# Autodesk Inventor assembly: Spidey
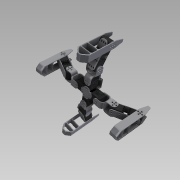
[picture p0: Inventor's stored thumbnail of the model, 180x180]
Saved by Autodesk Inventor 2014 (Build 180170000, 170)
## iProperties
Created: 2014-03-07
Part Number: Spidey
Document SubType Name: Assembly
Designer: Grégoire
Author: Grégoire
## Documents named in this file (10)
- C:\Users\Grégoire\Desktop\Spidey\3d\src\spidey.iam
- C:\Users\Grégoire\Desktop\Spidey\3d\src\models\motor.ipt
- C:\Users\Grégoire\Desktop\Spidey\3d\src\models\arm.ipt
- C:\Users\Grégoire\Desktop\Spidey\3d\src\models\counter_arm.ipt
- C:\Users\Grégoire\Desktop\Spidey\3d\src\parts\u.ipt
- C:\Users\Grégoire\Desktop\Spidey\3d\src\parts\side.ipt
- C:\Users\Grégoire\Desktop\Spidey\3d\src\parts\leg.ipt
- C:\Users\Grégoire\Desktop\Spidey\3d\src\parts\body.ipt
- C:\Users\Grégoire\Desktop\Spidey\3d\src\parts\body_with_fixations.ipt
- C:\Users\Grégoire\Desktop\Spidey\3d\src\parts\body_to_opencm.ipt
## Components (60 placed, 9 different names)
1. motor:4 — Placage:132, Placage:133, Placage:148, Placage:152
2. arm:4
3. counter_arm:4
4. u:3
5. u:4
6. motor:5
7. arm:5
8. counter_arm:5
9. side:3
10. side:4
11. motor:6
12. arm:6
13. counter_arm:6
14. leg:2
15. motor:7 — Placage:127, Placage:128, Placage:150, Placage:153, Placage:154
16. arm:7
17. counter_arm:7
18. u:5
19. u:6
20. motor:8
21. arm:8
22. counter_arm:8
23. side:5
24. side:6
25. motor:9
26. arm:9
27. counter_arm:9
28. leg:3
29. motor:10 — Placage:129, Placage:151, Placage:156, Placage:157
30. arm:10
31. counter_arm:10
32. u:7
33. u:8
34. motor:11
35. arm:11
36. counter_arm:11
37. side:7
38. side:8
39. motor:12
40. arm:12
41. counter_arm:12
42. leg:4
43. body:1 — Placage:127, Placage:128, Placage:129, Placage:130, Placage:131, Placage:132, Placage:133, Placage:148, Placage:165
44. body_with_fixations:1 — Placage:149, Placage:150, Placage:151, Placage:152, Placage:153, Placage:154, Placage:155, Placage:156, Placage:157, Placage:158, Placage:159, Placage:160, Placage:161, Placage:162, Placage:163
45. body_to_opencm:1 — Placage:158, Placage:162, Placage:163
46. body_to_opencm:2 — Placage:159, Placage:160, Placage:161
47. u:1 — Placage:7, Placage:8, Placage:9, Placage:14, Placage:15
48. u:2 — Placage:5, Placage:6, Placage:7, Placage:8, Placage:9, Placage:164
49. side:1 — Placage:19, Placage:20, Placage:21, Placage:26, Placage:27, Placage:28
50. side:2 — Placage:16, Placage:17, Placage:18
51. leg:1 — Placage:29, Placage:30
52. motor:1 — Placage:1, Placage:2, Placage:3, Placage:4, Placage:130, Placage:131, Placage:149, Placage:155
53. arm:1 — Placage:3, Placage:4, Placage:5, Placage:6
54. counter_arm:1 — Placage:1, Placage:2, Placage:164
55. motor:2 — Placage:16, Placage:17, Placage:18, Placage:19, Placage:20, Placage:21
56. arm:2 — Placage:15
57. counter_arm:2 — Placage:14
58. motor:3 — Placage:26, Placage:27, Placage:28
59. arm:3 — Placage:29, Placage:30
60. counter_arm:3
## Relationships (145: Mate 145)
- Placage:1 [Mate]: motor:1 ↔ counter_arm:1
- Placage:2 [Mate]: motor:1 ↔ counter_arm:1
- Placage:3 [Mate]: motor:1 ↔ arm:1
- Placage:4 [Mate]: motor:1 ↔ arm:1
- Placage:5 [Mate]: u:2 ↔ arm:1
- Placage:6 [Mate]: u:2 ↔ arm:1
- Placage:7 [Mate]: u:1 ↔ u:2
- Placage:8 [Mate]: u:1 ↔ u:2
- Placage:9 [Mate]: u:1 ↔ u:2
- [Mate]: motor:2 ↔ counter_arm:2
- [Mate]: motor:2 ↔ counter_arm:2
- [Mate]: motor:2 ↔ arm:2
- [Mate]: motor:2 ↔ arm:2
- Placage:14 [Mate]: u:1 ↔ counter_arm:2
- Placage:15 [Mate]: u:1 ↔ arm:2
- Placage:16 [Mate]: side:2 ↔ motor:2
- Placage:17 [Mate]: side:2 ↔ motor:2
- Placage:18 [Mate]: side:2 ↔ motor:2
- Placage:19 [Mate]: side:1 ↔ motor:2
- Placage:20 [Mate]: side:1 ↔ motor:2
- Placage:21 [Mate]: side:1 ↔ motor:2
- [Mate]: motor:3 ↔ counter_arm:3
- [Mate]: motor:3 ↔ counter_arm:3
- [Mate]: motor:3 ↔ arm:3
- [Mate]: motor:3 ↔ arm:3
- Placage:26 [Mate]: side:1 ↔ motor:3
- Placage:27 [Mate]: side:1 ↔ motor:3
- Placage:28 [Mate]: side:1 ↔ motor:3
- Placage:29 [Mate]: leg:1 ↔ arm:3
- Placage:30 [Mate]: leg:1 ↔ arm:3
- [Mate]: motor:4 ↔ counter_arm:4
- [Mate]: motor:4 ↔ counter_arm:4
- [Mate]: motor:4 ↔ arm:4
- [Mate]: motor:4 ↔ arm:4
- [Mate]: arm:4 ↔ u:4
- [Mate]: arm:4 ↔ u:4
- [Mate]: u:3 ↔ u:4
- [Mate]: u:3 ↔ u:4
- [Mate]: u:3 ↔ u:4
- [Mate]: motor:5 ↔ counter_arm:5
- [Mate]: motor:5 ↔ counter_arm:5
- [Mate]: motor:5 ↔ arm:5
- [Mate]: motor:5 ↔ arm:5
- [Mate]: u:3 ↔ counter_arm:5
- [Mate]: u:3 ↔ arm:5
- [Mate]: motor:5 ↔ side:4
- [Mate]: motor:5 ↔ side:4
- [Mate]: motor:5 ↔ side:4
- [Mate]: motor:5 ↔ side:3
- [Mate]: motor:5 ↔ side:3
- [Mate]: motor:5 ↔ side:3
- [Mate]: motor:6 ↔ counter_arm:6
- [Mate]: motor:6 ↔ counter_arm:6
- [Mate]: motor:6 ↔ arm:6
- [Mate]: motor:6 ↔ arm:6
- [Mate]: side:3 ↔ motor:6
- [Mate]: side:3 ↔ motor:6
- [Mate]: side:3 ↔ motor:6
- [Mate]: arm:6 ↔ leg:2
- [Mate]: arm:6 ↔ leg:2
- [Mate]: motor:7 ↔ counter_arm:7
- [Mate]: motor:7 ↔ counter_arm:7
- [Mate]: motor:7 ↔ arm:7
- [Mate]: motor:7 ↔ arm:7
- [Mate]: arm:7 ↔ u:6
- [Mate]: arm:7 ↔ u:6
- [Mate]: u:5 ↔ u:6
- [Mate]: u:5 ↔ u:6
- [Mate]: u:5 ↔ u:6
- [Mate]: motor:8 ↔ counter_arm:8
- [Mate]: motor:8 ↔ counter_arm:8
- [Mate]: motor:8 ↔ arm:8
- [Mate]: motor:8 ↔ arm:8
- [Mate]: u:5 ↔ counter_arm:8
- [Mate]: u:5 ↔ arm:8
- [Mate]: motor:8 ↔ side:6
- [Mate]: motor:8 ↔ side:6
- [Mate]: motor:8 ↔ side:6
- [Mate]: motor:8 ↔ side:5
- [Mate]: motor:8 ↔ side:5
- [Mate]: motor:8 ↔ side:5
- [Mate]: motor:9 ↔ counter_arm:9
- [Mate]: motor:9 ↔ counter_arm:9
- [Mate]: motor:9 ↔ arm:9
- [Mate]: motor:9 ↔ arm:9
- [Mate]: side:5 ↔ motor:9
- [Mate]: side:5 ↔ motor:9
- [Mate]: side:5 ↔ motor:9
- [Mate]: arm:9 ↔ leg:3
- [Mate]: arm:9 ↔ leg:3
- [Mate]: motor:10 ↔ counter_arm:10
- [Mate]: motor:10 ↔ counter_arm:10
- [Mate]: motor:10 ↔ arm:10
- [Mate]: motor:10 ↔ arm:10
- [Mate]: arm:10 ↔ u:8
- [Mate]: arm:10 ↔ u:8
- [Mate]: u:7 ↔ u:8
- [Mate]: u:7 ↔ u:8
- [Mate]: u:7 ↔ u:8
- [Mate]: motor:11 ↔ counter_arm:11
- [Mate]: motor:11 ↔ counter_arm:11
- [Mate]: motor:11 ↔ arm:11
- [Mate]: motor:11 ↔ arm:11
- [Mate]: u:7 ↔ counter_arm:11
- [Mate]: u:7 ↔ arm:11
- [Mate]: motor:11 ↔ side:8
- [Mate]: motor:11 ↔ side:8
- [Mate]: motor:11 ↔ side:8
- [Mate]: motor:11 ↔ side:7
- [Mate]: motor:11 ↔ side:7
- [Mate]: motor:11 ↔ side:7
- [Mate]: motor:12 ↔ counter_arm:12
- [Mate]: motor:12 ↔ counter_arm:12
- [Mate]: motor:12 ↔ arm:12
- [Mate]: motor:12 ↔ arm:12
- [Mate]: side:7 ↔ motor:12
- [Mate]: side:7 ↔ motor:12
- [Mate]: side:7 ↔ motor:12
- [Mate]: arm:12 ↔ leg:4
- [Mate]: arm:12 ↔ leg:4
- Placage:127 [Mate]: motor:7 ↔ body:1
- Placage:128 [Mate]: motor:7 ↔ body:1
- Placage:129 [Mate]: motor:10 ↔ body:1
- Placage:130 [Mate]: body:1 ↔ motor:1
- Placage:131 [Mate]: body:1 ↔ motor:1
- Placage:132 [Mate]: motor:4 ↔ body:1
- Placage:133 [Mate]: motor:4 ↔ body:1
- Placage:148 [Mate]: motor:4 ↔ body:1
- Placage:149 [Mate]: body_with_fixations:1 ↔ motor:1
- Placage:150 [Mate]: motor:7 ↔ body_with_fixations:1
- Placage:151 [Mate]: motor:10 ↔ body_with_fixations:1
- Placage:152 [Mate]: motor:4 ↔ body_with_fixations:1
- Placage:153 [Mate]: motor:7 ↔ body_with_fixations:1
- Placage:154 [Mate]: motor:7 ↔ body_with_fixations:1
- Placage:155 [Mate]: body_with_fixations:1 ↔ motor:1
- Placage:156 [Mate]: motor:10 ↔ body_with_fixations:1
- Placage:157 [Mate]: motor:10 ↔ body_with_fixations:1
- Placage:158 [Mate]: body_with_fixations:1 ↔ body_to_opencm:1
- Placage:159 [Mate]: body_with_fixations:1 ↔ body_to_opencm:2
- Placage:160 [Mate]: body_with_fixations:1 ↔ body_to_opencm:2
- Placage:161 [Mate]: body_with_fixations:1 ↔ body_to_opencm:2
- Placage:162 [Mate]: body_with_fixations:1 ↔ body_to_opencm:1
- Placage:163 [Mate]: body_with_fixations:1 ↔ body_to_opencm:1
- Placage:164 [Mate]: u:2 ↔ counter_arm:1
- Placage:165 [Mate]: body:1
## Named parameters: d25_d0 = 0 mm, d26_d1 = 0 mm, d27_d2 = 0 mm, d28_d3 = 0 mm, d37_d0 = 0 mm, d38_d1 = 0 mm, d39_d2 = 0 mm, d40_d3 = 0 mm, d52_d0 = 0 mm, d53_d1 = 0 mm, d54_d2 = 0 mm, d55_d3 = 0 mm, d56_d20 = 0 mm, d57_d21 = 0 mm, d58_d22 = 0 mm, d59_d23 = 0 mm, d60_d24 = 0 mm, d61_d25_d0 = 0 mm, d62_d26_d1 = 0 mm, d63_d27_d2 = 0 mm, d64_d28_d3 = 0 mm, d65_d29 = 0 mm, d66_d30 = 0 mm, d67_d31 = 0 mm, d68_d32 = 0 mm, d69_d33 = 0 mm, d70_d34 = 0 mm, d71_d35 = 0 mm, d72_d36 = 0 mm, d73_d37_d0 = 0 mm, d74_d38_d1 = 0 mm, d75_d39_d2 = 0 mm, d76_d40_d3 = 0 mm, d77_d41 = 0 mm, d78_d42 = 0 mm, d79_d43 = 0 mm, d80_d44 = 0 mm, d81_d45 = 0 mm, d82_d0 = 0 mm, d83_d1 = 0 mm, d84_d2 = 0 mm, d85_d3 = 0 mm, d86_d20 = 0 mm, d87_d21 = 0 mm, d88_d22 = 0 mm, d89_d23 = 0 mm, d90_d24 = 0 mm, d91_d25_d0 = 0 mm, d92_d26_d1 = 0 mm, d93_d27_d2 = 0 mm, d94_d28_d3 = 0 mm, d95_d29 = 0 mm, d96_d30 = 0 mm, d97_d31 = 0 mm, d98_d32 = 0 mm, d99_d33 = 0 mm, d100_d34 = 0 mm, d101_d35 = 0 mm, d102_d36 = 0 mm, d103_d37_d0 = 0 mm, d104_d38_d1 = 0 mm, d105_d39_d2 = 0 mm, d106_d40_d3 = 0 mm, d107_d41 = 0 mm, d108_d42 = 0 mm, d109_d43 = 0 mm, d110_d44 = 0 mm, d111_d45 = 0 mm, d112_d0 = 0 mm, d113_d1 = 0 mm, d114_d2 = 0 mm, d115_d3 = 0 mm, d116_d20 = 0 mm, d117_d21 = 0 mm, d118_d22 = 0 mm, d119_d23 = 0 mm, d120_d24 = 0 mm, d121_d25_d0 = 0 mm, d122_d26_d1 = 0 mm, d123_d27_d2 = 0 mm, d124_d28_d3 = 0 mm, d125_d29 = 0 mm, d126_d30 = 0 mm, d127_d31 = 0 mm, d128_d32 = 0 mm, d129_d33 = 0 mm, d130_d34 = 0 mm, d131_d35 = 0 mm, d132_d36 = 0 mm, d133_d37_d0 = 0 mm, d134_d38_d1 = 0 mm, d135_d39_d2 = 0 mm, d136_d40_d3 = 0 mm, d137_d41 = 0 mm, d138_d42 = 0 mm, d139_d43 = 0 mm, d140_d44 = 0 mm, d141_d45 = 0 mm
